# Autodesk Inventor assembly: singleModule
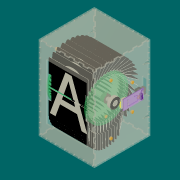
[picture p0: Inventor's stored thumbnail of the model, 180x180]
Saved by Autodesk Inventor 2016 (Build 200138000, 138)
## iProperties
Created: 2015-10-05
Part Number: singleModule
Document SubType Name: Assembly
Designer: Sawaiz
Author: Sawaiz
## Documents named in this file (7)
- C:\Users\sawaiz\oneDrive\projects\splitFlapDisplay\singleModule.iam
- C:\Users\sawaiz\oneDrive\projects\splitFlapDisplay\frame\frame.iam
- C:\Users\sawaiz\oneDrive\projects\splitFlapDisplay\spool\cardSpool.iam
- C:\Users\sawaiz\oneDrive\projects\splitFlapDisplay\drive\drive.iam
- C:\Users\sawaiz\oneDrive\projects\splitFlapDisplay\drive\centeralShaft.ipt
- C:\Users\sawaiz\oneDrive\projects\splitFlapDisplay\drive\belt.ipt
- C:\Users\sawaiz\oneDrive\projects\splitFlapDisplay\parameters.xlsx
## Components (5 placed, 5 different names)
1. cardSpool:1 [sub-assembly] — Angle:3, Mate:32, Mate:34, Mate:35
2. drive:1 [sub-assembly] — Mate:28, Mate:29, Angle:2, Mate:33
3. frame:1 [sub-assembly] — Mate:25, Angle:2, Flush:2, Angle:3, Mate:32, Mate:33, Angle:4
4. centeralShaft:1 — Mate:25, Flush:2, Mate:35
5. belt:1 — Mate:28, Mate:29, Mate:34, Angle:4
## Relationships (11: Mate 7, Angle 3, Flush 1)
- Mate:25: frame:1 ↔ centeralShaft:1
- Mate:28: drive:1 ↔ belt:1
- Mate:29 (1 mm): drive:1 ↔ belt:1
- Angle:2 (0 deg): drive:1 ↔ frame:1
- Flush:2: frame:1 ↔ centeralShaft:1
- Angle:3 (0 deg): cardSpool:1 ↔ frame:1
- Mate:32 (0.5 mm): cardSpool:1 ↔ frame:1
- Mate:33: drive:1 ↔ frame:1
- Mate:34: cardSpool:1 ↔ belt:1
- Mate:35: cardSpool:1 ↔ centeralShaft:1
- Angle:4 (-37.21 deg): frame:1 ↔ belt:1
## Named parameters: height = 180 mm, width = 120 mm, depth = 120 mm, materialThickness = 3.175 mm, laserKerf = 0.12 mm, spoolDiameter = 90 mm, cardPinDiameter = 3 mm, cardNumber = 40, centeralShaftDiameter = 8 mm, cardWidth = 85.6 mm, cardHeight = 53.98 mm, cardThickness = 0.76 mm, cardFillet = 2.88 mm, cardCutoutHeight = 20 mm, cardClearence = 0.5 mm, spoolHubDiameter = 20 mm, bearingOd = 22 mm, bearingWidth = 8 mm, axleHeight = 95 mm, nutTrapDepth = 2.5 mm, nutTrapwidth = 5.5 mm, nutTrapClearence = 2 mm, beltLength = 240 mm, magnetDiameter = 6 mm, magnetLength = 3 mm, magnetProtusion = 0.25 mm, notchWidth = 10 mm, spoolThickness = 5.588 mm
